# Autodesk Inventor assembly: driven wheel assembly right
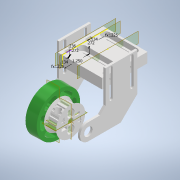
[picture p0: Inventor's stored thumbnail of the model, 180x180]
Saved by Autodesk Inventor 2020 (Build 240168000, 168)
## iProperties
Created: 2020-01-25
Part Number: driven wheel assembly right
Document SubType Name: Assembly
Designer: ball
Author: ball
## Documents named in this file (4)
- D:\FTC8863\2019 Robot\Collection\Intake\driven wheel assembly right.iam
- D:\FTC8863\2019 Robot\Collection\Intake\driven wheel mount to xrail.ipt
- D:\FTC8863\2019 Robot\general robot componets\pulley .25 in + wheel.2.iam
- D:\FTC8863\2019 Robot\Collection\Intake\driven wheel arm angled.ipt
## Components (4 placed, 3 different names)
1. driven wheel mount to xrail:1 — Mate:5, Mate:6, Flush:5, Flush:6
2. driven wheel arm angled:1 — Mate:5, Flush:3, Flush:4, Flush:5, Flush:6
3. pulley .25 in + wheel.2:1 [sub-assembly] — Mate:7, Mate:8
4. driven wheel arm angled:2 — Mate:6, Flush:3, Flush:4, Mate:7, Mate:8
## Relationships (8: Mate 4, Flush 4)
- Mate:5: driven wheel mount to xrail:1 ↔ driven wheel arm angled:1
- Mate:6: driven wheel mount to xrail:1 ↔ driven wheel arm angled:2
- Flush:3: driven wheel arm angled:1 ↔ driven wheel arm angled:2
- Flush:4: driven wheel arm angled:1 ↔ driven wheel arm angled:2
- Mate:7: pulley .25 in + wheel.2:1 ↔ driven wheel arm angled:2
- Mate:8 (6.35 mm): pulley .25 in + wheel.2:1 ↔ driven wheel arm angled:2
- Flush:5 (-1.4986 mm): driven wheel mount to xrail:1 ↔ driven wheel arm angled:1
- Flush:6 (10.16 mm): driven wheel mount to xrail:1 ↔ driven wheel arm angled:1
